# Autodesk Inventor assembly: FirstTryAssembly(kopia)
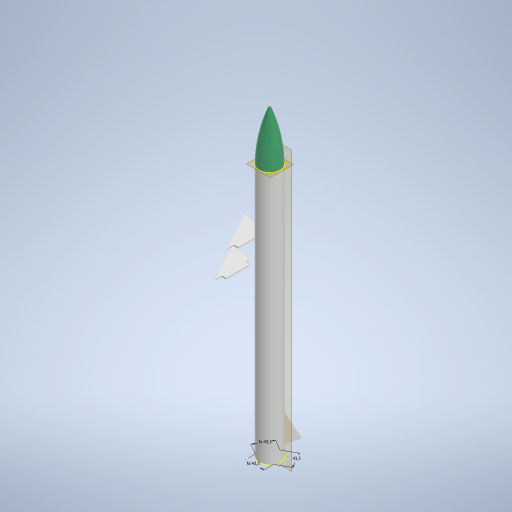
[picture p0: Inventor's stored thumbnail of the model, 512x512]
Saved by Autodesk Inventor 2023.2 (Build 272271000, 271)
## iProperties
Created: 2022-12-18
Part Number: FirstTryAssembly(kopia)
Document SubType Name: Assembly
Designer: Admin
Author: Admin
## Documents named in this file (8)
- C:\Users\Admin\Desktop\Rakietka\FirstTryAssembly(kopia).iam
- C:\Users\Admin\Desktop\Rakietka\Korpus.ipt
- C:\Users\Admin\Desktop\Rakietka\EngineBlock.ipt
- C:\Users\Admin\Desktop\Rakietka\nose-cone.ipt
- C:\Users\Admin\Desktop\Rakietka\PrzegrodaNaElektronike.ipt
- C:\Users\Admin\Desktop\Rakietka\RuraWewnetrznaSilnik.ipt
- C:\Users\Admin\Desktop\Rakietka\Stateczniki.ipt
- C:\Users\Admin\Desktop\Rakietka\CenterRing.ipt
## Components (11 placed, 7 different names)
1. Korpus:1 — Mate:3, Mate:4, Mate:5, Mate:6, Mate:7, Mate:8, Flush:2, Mate:9, Flush:3, Mate:10, Flush:4, Mate:11, Flush:5, Mate:12, Mate:13, Flush:6
2. EngineBlock:1 — Mate:7, Flush:1
3. nose-cone:1 — Mate:12
4. PrzegrodaNaElektronike:1 — Mate:11, Flush:5
5. RuraWewnetrznaSilnik:1 — Mate:3, Mate:6, Flush:1
6. Stateczniki:1 — Mate:4, Mate:5, Mate:13, Flush:6
7. Stateczniki:2
8. Stateczniki:3
9. PrzegrodaNaElektronike:2 — Mate:10, Flush:4
10. CenterRing:1 — Mate:9, Flush:3
11. CenterRing:2 — Mate:8, Flush:2
## Relationships (17: Mate 11, Flush 6)
- Mate:3: Korpus:1 ↔ RuraWewnetrznaSilnik:1
- Mate:4: Korpus:1 ↔ Stateczniki:1
- Mate:5: Korpus:1 ↔ Stateczniki:1
- Mate:6: Korpus:1 ↔ RuraWewnetrznaSilnik:1
- Mate:7: Korpus:1 ↔ EngineBlock:1
- Flush:1 (5 mm): EngineBlock:1 ↔ RuraWewnetrznaSilnik:1
- Mate:8: Korpus:1 ↔ CenterRing:2
- Flush:2 (17 mm): Korpus:1 ↔ CenterRing:2
- Mate:9: Korpus:1 ↔ CenterRing:1
- Flush:3 (75 mm): Korpus:1 ↔ CenterRing:1
- Mate:10: Korpus:1 ↔ PrzegrodaNaElektronike:2
- Flush:4 (407 mm): Korpus:1 ↔ PrzegrodaNaElektronike:2
- Mate:11: Korpus:1 ↔ PrzegrodaNaElektronike:1
- Flush:5 (357 mm): Korpus:1 ↔ PrzegrodaNaElektronike:1
- Mate:12: Korpus:1 ↔ nose-cone:1
- Mate:13: Korpus:1 ↔ Stateczniki:1
- Flush:6 (-10.5 mm): Korpus:1 ↔ Stateczniki:1
